# Autodesk Inventor assembly: gate_or
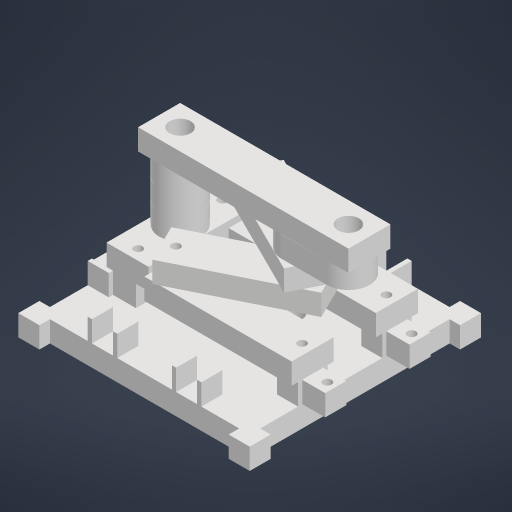
[picture p0: Inventor's stored thumbnail of the model, 512x512]
Saved by Autodesk Inventor 2024.3 (Build 283343000, 343)
## iProperties
Created: 2024-09-29
Part Number: gate_or
Document SubType Name: Assembly
Designer: sam
Author: sam
## Documents named in this file (10)
- N:\Cad\computer\gates\gate_or.iam
- N:\Cad\computer\gates\base.ipt
- N:\Cad\computer\gates\block.ipt
- N:\Cad\computer\gates\link_small.ipt
- N:\Cad\computer\gates\bar.ipt
- N:\Cad\computer\gates\extender.ipt
- N:\Cad\computer\gates\connector_small.ipt
- N:\Cad\computer\gates\extender_large.ipt
- N:\Cad\computer\gates\spacer_small.ipt
- N:\Cad\computer\gates\spacer.ipt
## Components (15 placed, 9 different names)
1. base:1 — Mate:1, Mate:2, Mate:3, Mate:4, Mate:5, Mate:6
2. block:1 — Mate:5, Mate:6, Mate:11, Flush:1, Mate:12
3. block:2 — Mate:1, Mate:2, Mate:13, Mate:15, Flush:2
4. block:3 — Mate:3, Mate:4, Mate:14, Mate:16, Flush:3
5. link_small:1 — Mate:8, Mate:19, Mate:23, Mate:24, Mate:33
6. link_small:2 — Mate:8, Mate:17, Mate:21
7. bar:3 — Mate:11, Flush:1, Mate:12, Mate:25, Mate:26, Flush:7
8. extender:1 — Mate:14, Mate:16, Flush:3, Mate:22
9. extender:2 — Mate:13, Mate:15, Mate:17, Flush:2, Mate:21
10. connector_small:1 — Mate:19, Mate:33, Mate:34
11. extender_large:1 — Mate:31, Mate:32, Flush:7, Mate:34
12. spacer_small:1 — Mate:22, Mate:23, Mate:24
13. spacer:1 — Mate:25, Mate:26, Mate:27, Mate:28
14. spacer:2 — Mate:27, Mate:28, Mate:29, Mate:30
15. spacer:3 — Mate:29, Mate:30, Mate:31, Mate:32
## Relationships (34: Mate 30, Flush 4)
- Mate:1: base:1 ↔ block:2
- Mate:2: base:1 ↔ block:2
- Mate:3: base:1 ↔ block:3
- Mate:4: base:1 ↔ block:3
- Mate:5: base:1 ↔ block:1
- Mate:6: base:1 ↔ block:1
- [Mate]: link_small:1 ↔ link_small:2
- Mate:8: link_small:1 ↔ link_small:2
- Mate:11: block:1 ↔ bar:3
- Flush:1: block:1 ↔ bar:3
- Mate:12: block:1 ↔ bar:3
- Mate:13: block:2 ↔ extender:2
- Mate:14: block:3 ↔ extender:1
- Mate:15: block:2 ↔ extender:2
- Mate:16: block:3 ↔ extender:1
- Mate:17: link_small:2 ↔ extender:2
- Flush:2 (5.5 mm): block:2 ↔ extender:2
- Flush:3 (5.5 mm): block:3 ↔ extender:1
- Mate:19: link_small:1 ↔ connector_small:1
- Mate:21: link_small:2 ↔ extender:2
- Mate:22: extender:1 ↔ spacer_small:1
- Mate:23: link_small:1 ↔ spacer_small:1
- Mate:24: link_small:1 ↔ spacer_small:1
- Mate:25: bar:3 ↔ spacer:1
- Mate:26: bar:3 ↔ spacer:1
- Mate:27: spacer:1 ↔ spacer:2
- Mate:28: spacer:1 ↔ spacer:2
- Mate:29: spacer:2 ↔ spacer:3
- Mate:30: spacer:2 ↔ spacer:3
- Mate:31: extender_large:1 ↔ spacer:3
- Mate:32: extender_large:1 ↔ spacer:3
- Mate:33: link_small:1 ↔ connector_small:1
- Flush:7: bar:3 ↔ extender_large:1
- Mate:34: connector_small:1 ↔ extender_large:1
